# Autodesk Inventor assembly: standoff_brace
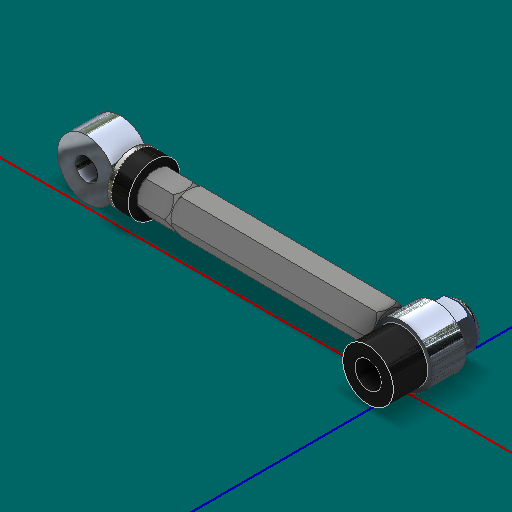
[picture p0: Inventor's stored thumbnail of the model, 512x512]
Saved by Autodesk Inventor 2025 (Build 290162000, 162)
## iProperties
Created: 2024-08-17
Part Number: standoff_brace
Document SubType Name: Assembly
Designer: averey
Author: averey
## Documents named in this file (11)
- C:\Users\avere\vex_robotics_high_stakes\hardware\cad\ATLAS\chassis\standoff_brace.iam
- C:\Users\avere\vex_robotics_high_stakes\hardware\cad\VEX-CAD-Inventor\Motion\Shaft LS\Shaft Collar ipts\Shaft Collar No Screw.ipt
- C:\Users\avere\vex_robotics_high_stakes\hardware\cad\VEX-CAD-Inventor\Structure\Standoff\Standoff .25.ipt
- C:\Users\avere\vex_robotics_high_stakes\hardware\cad\VEX-CAD-Inventor\Structure\Standoff.ipt
- C:\Users\avere\vex_robotics_high_stakes\hardware\cad\VEX-CAD-Inventor\Structure\Standoff\Standoff 1.50.ipt
- C:\Users\avere\vex_robotics_high_stakes\hardware\cad\VEX-CAD-Inventor\Motion\Spacers\Spacer Nylon .375 OD\NSpacer .375 OD x .125.ipt
- C:\Users\avere\vex_robotics_high_stakes\hardware\cad\VEX-CAD-Inventor\Motion\Spacers\Spacer Nylon .375 OD.ipt
- C:\Users\avere\vex_robotics_high_stakes\hardware\cad\VEX-CAD-Inventor\Motion\Spacers\Washer Steel\SWasher .375 OD x .031250.ipt
- C:\Users\avere\vex_robotics_high_stakes\hardware\cad\VEX-CAD-Inventor\Motion\Spacers\Washer Steel.ipt
- C:\Users\avere\vex_robotics_high_stakes\hardware\cad\VEX-CAD-Inventor\Motion\Spacers\Spacer Nylon .375 OD\NSpacer .375 OD x .250.ipt
- C:\Users\avere\vex_robotics_high_stakes\hardware\cad\VEX-CAD-Inventor\Structure\Hardware\Nut Thin Nylock.ipt
## Components (8 placed, 7 different names)
1. Shaft Collar No Screw:1
2. Shaft Collar No Screw:2 — Mate:2, Mate:4, Insert:5, Insert:6
3. Standoff .25:1
4. Standoff 1.50:2 — Angle:1, Mate:4
5. NSpacer .375 OD x .125:1
6. SWasher .375 OD x .031250:1
7. NSpacer .375 OD x .250:2 — Insert:5
8. Nut Thin Nylock:1 — Insert:6
## Relationships (9: Insert 6, Mate 2, Angle 1)
- [Insert]: Standoff .25:1 ↔ Standoff 1.50:2
- [Insert]: NSpacer .375 OD x .125:1 ↔ SWasher .375 OD x .031250:1
- [Insert]: Standoff .25:1 ↔ NSpacer .375 OD x .125:1
- [Insert]: Shaft Collar No Screw:1 ↔ SWasher .375 OD x .031250:1
- Mate:2: Shaft Collar No Screw:2
- Angle:1 (0 deg): Standoff 1.50:2
- Mate:4: Shaft Collar No Screw:2 ↔ Standoff 1.50:2
- Insert:5: Shaft Collar No Screw:2 ↔ NSpacer .375 OD x .250:2
- Insert:6: Shaft Collar No Screw:2 ↔ Nut Thin Nylock:1
